# Autodesk Inventor assembly: Test_khung_xe
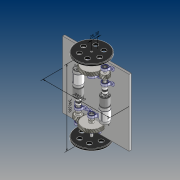
[picture p0: Inventor's stored thumbnail of the model, 180x180]
Saved by Autodesk Inventor 2021 (Build 250183000, 183)
## iProperties
Created: 2024-03-25
Part Number: Test_khung_xe
Document SubType Name: Assembly
Designer: Admin
Author: Admin
## Documents named in this file (3)
- C:\Users\Admin\Desktop\DO_AN_TOT_NGHIEP_2024\Mechanical\Design_in_3D\Version_1\Example\Test_khung_xe.iam
- C:\Users\Admin\Desktop\DO_AN_TOT_NGHIEP_2024\Mechanical\Design_in_3D\Version_1\06_Tam_de_01.ipt
- C:\Users\Admin\Desktop\DO_AN_TOT_NGHIEP_2024\Mechanical\Design_in_3D\Version_1\000ASS_Bo_banh_xe_03.iam
## Components (3 placed, 2 different names)
1. 06_Tam_de_01:1 — Mate:1, Mate:2, Angle:1, Mate:4, Mate:5
2. 000ASS_Bo_banh_xe_03:1 [sub-assembly] — Mate:1, Mate:3, Mate:4
3. 000ASS_Bo_banh_xe_03:2 [sub-assembly] — Mate:2, Angle:1, Mate:3, Mate:5
## Relationships (6: Mate 5, Angle 1)
- Mate:1: 06_Tam_de_01:1 ↔ 000ASS_Bo_banh_xe_03:1
- Mate:2: 06_Tam_de_01:1 ↔ 000ASS_Bo_banh_xe_03:2
- Angle:1 (180 deg): 06_Tam_de_01:1 ↔ 000ASS_Bo_banh_xe_03:2
- Mate:3: 000ASS_Bo_banh_xe_03:1 ↔ 000ASS_Bo_banh_xe_03:2
- Mate:4 (10 mm): 06_Tam_de_01:1 ↔ 000ASS_Bo_banh_xe_03:1
- Mate:5 (10 mm): 06_Tam_de_01:1 ↔ 000ASS_Bo_banh_xe_03:2
